# Autodesk Inventor assembly: plotter_new
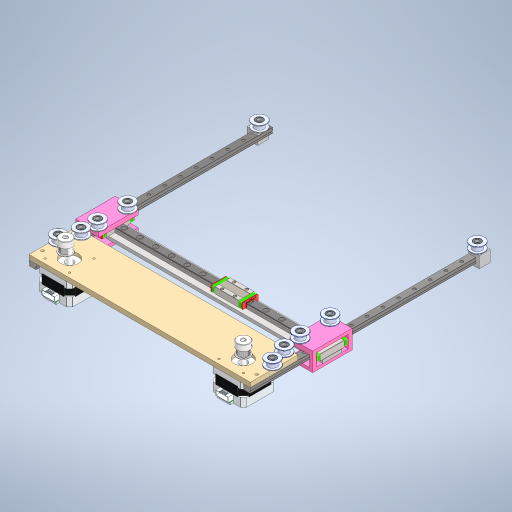
[picture p0: Inventor's stored thumbnail of the model, 512x512]
Saved by Autodesk Inventor 2023.1 (Build 271208000, 208)
## iProperties
Created: 2025-12-22
Part Number: plotter_new
Document SubType Name: Assembly
Designer: DELL
Author: DELL
## Documents named in this file (15)
- C:\Users\DELL\reposGitHub\VSOSH25-26\models\plotter\plotter_new.iam
- C:\Users\DELL\reposGitHub\VSOSH25-26\models\import\MGN9-H.ipt
- C:\Users\DELL\reposGitHub\VSOSH25-26\models\actuator\рельса.ipt
- C:\Users\DELL\reposGitHub\VSOSH25-26\models\import\Stepper motor Nema 17 (17HS2408).ipt
- C:\Users\DELL\reposGitHub\VSOSH25-26\models\actuator\центр_рейка.ipt
- C:\Users\DELL\reposGitHub\VSOSH25-26\models\actuator\креп_мотора.ipt
- C:\Users\DELL\reposGitHub\VSOSH25-26\models\import\Ролик с резьбой GT2 на моторы.ipt
- C:\Users\DELL\reposGitHub\VSOSH25-26\models\import\Сборка ролик с подшипником.ipt
- C:\Users\DELL\reposGitHub\VSOSH25-26\models\plotter\креп_центр_ролик.ipt
- C:\Users\DELL\reposGitHub\VSOSH25-26\models\plotter\ограничитель.ipt
- C:\Users\DELL\reposGitHub\VSOSH25-26\models\actuator\рельса_центр.ipt
- C:\Users\DELL\reposGitHub\VSOSH25-26\models\import\Ролик с резьбой GT2 на моторы_MIR1.ipt
- C:\Users\DELL\reposGitHub\VSOSH25-26\models\import\Сборка ролик с подшипником_MIR3.ipt
- C:\Users\DELL\reposGitHub\VSOSH25-26\models\plotter\креп_центр_ролик_MIR.ipt
- C:\Users\DELL\reposGitHub\VSOSH25-26\models\plotter\ограничитель_MIR.ipt
## Components (26 placed, 14 different names)
1. рельса:1 — Совмещение:1, Совмещение:5, Совмещение:6, Совмещение:11, Заподлицо:7, Заподлицо:8, Совмещение:12, Заподлицо:9, Совмещение:22, Совмещение:25, Заподлицо:20, Совмещение:26
2. MGN9-H:1 — Совмещение:5, Совмещение:6, Совмещение:23, Заподлицо:19, Совмещение:47, Совмещение:48
3. Stepper motor Nema 17 (17HS2408):2 — Заподлицо:7, Заподлицо:8, Совмещение:12, Заподлицо:18, Совмещение:18
4. рельса:2 — Заподлицо:13, Заподлицо:14, Заподлицо:15, Совмещение:15, Совмещение:16, Заподлицо:16, Совмещение:50, Совмещение:51
5. MGN9-H:2 — Совмещение:36, Заподлицо:22, Совмещение:46, Совмещение:49
6. Stepper motor Nema 17 (17HS2408):3 — Заподлицо:14, Заподлицо:15, Совмещение:15
7. креп_мотора:1 — Заподлицо:18, Совмещение:19, Совмещение:53, Совмещение:54, Совмещение:55, Совмещение:56, Совмещение:57, Совмещение:58, Совмещение:59
8. Ролик с резьбой GT2 на моторы:1 — Совмещение:18, Совмещение:19
9. Сборка ролик с подшипником:1 — Совмещение:54, Совмещение:55
10. креп_центр_ролик:1 — Совмещение:22, Совмещение:23, Заподлицо:19, Совмещение:31, Совмещение:32, Совмещение:33, Совмещение:34
11. ограничитель:1 — Совмещение:25, Заподлицо:20, Совмещение:26, Совмещение:27, Совмещение:28
12. Сборка ролик с подшипником:2 — Совмещение:27, Совмещение:28
13. Сборка ролик с подшипником:3 — Совмещение:53
14. Сборка ролик с подшипником:4 — Совмещение:33, Совмещение:34
15. Сборка ролик с подшипником:5 — Совмещение:31, Совмещение:32
16. рельса_центр:1 — Совмещение:36, Совмещение:37, Совмещение:38, Совмещение:52, Заподлицо:23
17. MGN9-H:3 — Совмещение:37, Совмещение:38
18. Ролик с резьбой GT2 на моторы_MIR1:1
19. Сборка ролик с подшипником_MIR3:1 — Совмещение:58, Совмещение:59
20. креп_центр_ролик_MIR:1 — Совмещение:41, Совмещение:42, Совмещение:43, Совмещение:44, Заподлицо:22, Совмещение:46
21. ограничитель_MIR:1 — Совмещение:39, Совмещение:40, Совмещение:50, Совмещение:51
22. Сборка ролик с подшипником_MIR3:2 — Совмещение:39, Совмещение:40
23. Сборка ролик с подшипником_MIR3:3 — Совмещение:56, Совмещение:57
24. Сборка ролик с подшипником_MIR3:4 — Совмещение:41, Совмещение:42
25. Сборка ролик с подшипником_MIR3:5 — Совмещение:43, Совмещение:44
26. центр_рейка:1 — Совмещение:47, Совмещение:48, Совмещение:49, Совмещение:52, Заподлицо:23
## Relationships (56: Mate 44, Flush 12)
- Совмещение:1 [Mate] (131.4 mm): рельса:1
- Совмещение:5 [Mate]: рельса:1 ↔ MGN9-H:1
- Совмещение:6 [Mate] (-0.2 mm): рельса:1 ↔ MGN9-H:1
- Совмещение:11 [Mate]: рельса:1
- Заподлицо:7 [Flush]: рельса:1 ↔ Stepper motor Nema 17 (17HS2408):2
- Заподлицо:8 [Flush]: рельса:1 ↔ Stepper motor Nema 17 (17HS2408):2
- Совмещение:12 [Mate]: рельса:1 ↔ Stepper motor Nema 17 (17HS2408):2
- Заподлицо:9 [Flush] (150 mm): рельса:1
- [Mate]: рельса:2 ↔ MGN9-H:2
- [Mate] (-0.2 mm): рельса:2 ↔ MGN9-H:2
- Заподлицо:13 [Flush] (-150 mm): рельса:2
- Заподлицо:14 [Flush]: рельса:2 ↔ Stepper motor Nema 17 (17HS2408):3
- Заподлицо:15 [Flush]: рельса:2 ↔ Stepper motor Nema 17 (17HS2408):3
- Совмещение:15 [Mate]: рельса:2 ↔ Stepper motor Nema 17 (17HS2408):3
- Совмещение:16 [Mate]: рельса:2
- Заподлицо:16 [Flush] (131.4 mm): рельса:2
- Заподлицо:18 [Flush]: Stepper motor Nema 17 (17HS2408):2 ↔ креп_мотора:1
- Совмещение:18 [Mate]: Stepper motor Nema 17 (17HS2408):2 ↔ Ролик с резьбой GT2 на моторы:1
- Совмещение:19 [Mate] (5 mm): креп_мотора:1 ↔ Ролик с резьбой GT2 на моторы:1
- Совмещение:22 [Mate]: рельса:1 ↔ креп_центр_ролик:1
- Совмещение:23 [Mate]: MGN9-H:1 ↔ креп_центр_ролик:1
- Заподлицо:19 [Flush]: MGN9-H:1 ↔ креп_центр_ролик:1
- Совмещение:25 [Mate]: рельса:1 ↔ ограничитель:1
- Заподлицо:20 [Flush]: рельса:1 ↔ ограничитель:1
- Совмещение:26 [Mate]: рельса:1 ↔ ограничитель:1
- Совмещение:27 [Mate]: ограничитель:1 ↔ Сборка ролик с подшипником:2
- Совмещение:28 [Mate]: ограничитель:1 ↔ Сборка ролик с подшипником:2
- Совмещение:31 [Mate]: креп_центр_ролик:1 ↔ Сборка ролик с подшипником:5
- Совмещение:32 [Mate]: креп_центр_ролик:1 ↔ Сборка ролик с подшипником:5
- Совмещение:33 [Mate]: креп_центр_ролик:1 ↔ Сборка ролик с подшипником:4
- Совмещение:34 [Mate]: креп_центр_ролик:1 ↔ Сборка ролик с подшипником:4
- Совмещение:36 [Mate]: MGN9-H:2 ↔ рельса_центр:1
- Совмещение:37 [Mate]: рельса_центр:1 ↔ MGN9-H:3
- Совмещение:38 [Mate] (0.2 mm): рельса_центр:1 ↔ MGN9-H:3
- Совмещение:39 [Mate]: ограничитель_MIR:1 ↔ Сборка ролик с подшипником_MIR3:2
- Совмещение:40 [Mate]: ограничитель_MIR:1 ↔ Сборка ролик с подшипником_MIR3:2
- Совмещение:41 [Mate]: креп_центр_ролик_MIR:1 ↔ Сборка ролик с подшипником_MIR3:4
- Совмещение:42 [Mate]: креп_центр_ролик_MIR:1 ↔ Сборка ролик с подшипником_MIR3:4
- Совмещение:43 [Mate]: креп_центр_ролик_MIR:1 ↔ Сборка ролик с подшипником_MIR3:5
- Совмещение:44 [Mate]: креп_центр_ролик_MIR:1 ↔ Сборка ролик с подшипником_MIR3:5
- Заподлицо:22 [Flush]: MGN9-H:2 ↔ креп_центр_ролик_MIR:1
- Совмещение:46 [Mate]: MGN9-H:2 ↔ креп_центр_ролик_MIR:1
- Совмещение:47 [Mate]: MGN9-H:1 ↔ центр_рейка:1
- Совмещение:48 [Mate]: MGN9-H:1 ↔ центр_рейка:1
- Совмещение:49 [Mate]: MGN9-H:2 ↔ центр_рейка:1
- Совмещение:50 [Mate]: рельса:2 ↔ ограничитель_MIR:1
- Совмещение:51 [Mate]: рельса:2 ↔ ограничитель_MIR:1
- Совмещение:52 [Mate]: рельса_центр:1 ↔ центр_рейка:1
- Заподлицо:23 [Flush] (-7.5 mm): рельса_центр:1 ↔ центр_рейка:1
- Совмещение:53 [Mate]: креп_мотора:1 ↔ Сборка ролик с подшипником:3
- Совмещение:54 [Mate]: креп_мотора:1 ↔ Сборка ролик с подшипником:1
- Совмещение:55 [Mate]: креп_мотора:1 ↔ Сборка ролик с подшипником:1
- Совмещение:56 [Mate]: креп_мотора:1 ↔ Сборка ролик с подшипником_MIR3:3
- Совмещение:57 [Mate]: креп_мотора:1 ↔ Сборка ролик с подшипником_MIR3:3
- Совмещение:58 [Mate]: креп_мотора:1 ↔ Сборка ролик с подшипником_MIR3:1
- Совмещение:59 [Mate]: креп_мотора:1 ↔ Сборка ролик с подшипником_MIR3:1
## Named parameters: d34_d9 = 0 mm, d35_d10 = -0.2 mm
